# Autodesk Inventor assembly: NASA-20-EBOX-EXT-01
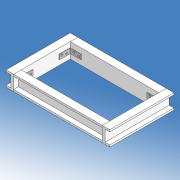
[picture p0: Inventor's stored thumbnail of the model, 180x180]
Saved by Autodesk Inventor 2020 (Build 240168000, 168)
## iProperties
Created: 2019-10-09
Part Number: NASA-20-EBOX-EXT-01
Document SubType Name: Assembly
Designer: mpark
Author: mpark
## Documents named in this file (4)
- C:\Users\mpark\Documents\NASA20\Inventor Files\NASA-20\NASA-20\E-Box\NASA-20-EBOX-EXT-01.iam
- C:\Users\mpark\Documents\NASA20\Inventor Files\NASA-20\NASA-20\E-Box\NASA-20-EBOX-EXTC-01.ipt
- C:\Users\mpark\Documents\NASA20\Inventor Files\NASA-20\NASA-20\E-Box\NASA-20-EBOX-SEXTC-01.ipt
- C:\Users\mpark\Documents\NASA20\Inventor Files\NASA-20\NASA-20\E-Box\1556A630_BRACKET.ipt
## Components (8 placed, 3 different names)
1. NASA-20-EBOX-EXTC-01:1 — Flush:1, Flush:2, Flush:5, Mate:1, Mate:2, Flush:8, Mate:8, Mate:9, Flush:9
2. NASA-20-EBOX-EXTC-01:2 — Flush:1, Flush:2, Flush:3, Flush:4, Flush:5, Flush:6, Flush:7, Mate:11, Mate:12
3. NASA-20-EBOX-SEXTC-01:1 — Flush:4, Mate:2, Flush:7, Mate:3, Mate:13
4. NASA-20-EBOX-SEXTC-01:2 — Flush:3, Mate:1, Flush:6, Flush:8, Mate:4, Mate:10
5. 1556A630_BRACKET:1 — Mate:3, Mate:8, Flush:9, Flush:10, Flush:11
6. 1556A630_BRACKET:4 — Mate:4, Mate:9, Flush:10
7. 1556A630_BRACKET:5 — Mate:10, Mate:11, Flush:12
8. 1556A630_BRACKET:6 — Mate:12, Mate:13, Flush:11, Flush:12
## Relationships (22: Flush 12, Mate 10)
- Flush:1: NASA-20-EBOX-EXTC-01:1 ↔ NASA-20-EBOX-EXTC-01:2
- Flush:2: NASA-20-EBOX-EXTC-01:1 ↔ NASA-20-EBOX-EXTC-01:2
- Flush:3: NASA-20-EBOX-EXTC-01:2 ↔ NASA-20-EBOX-SEXTC-01:2
- Flush:4: NASA-20-EBOX-EXTC-01:2 ↔ NASA-20-EBOX-SEXTC-01:1
- Flush:5: NASA-20-EBOX-EXTC-01:1 ↔ NASA-20-EBOX-EXTC-01:2
- Mate:1: NASA-20-EBOX-EXTC-01:1 ↔ NASA-20-EBOX-SEXTC-01:2
- Mate:2: NASA-20-EBOX-EXTC-01:1 ↔ NASA-20-EBOX-SEXTC-01:1
- Flush:6: NASA-20-EBOX-EXTC-01:2 ↔ NASA-20-EBOX-SEXTC-01:2
- Flush:7: NASA-20-EBOX-EXTC-01:2 ↔ NASA-20-EBOX-SEXTC-01:1
- Flush:8: NASA-20-EBOX-EXTC-01:1 ↔ NASA-20-EBOX-SEXTC-01:2
- Mate:3: NASA-20-EBOX-SEXTC-01:1 ↔ 1556A630_BRACKET:1
- Mate:4: NASA-20-EBOX-SEXTC-01:2 ↔ 1556A630_BRACKET:4
- Mate:8: NASA-20-EBOX-EXTC-01:1 ↔ 1556A630_BRACKET:1
- Mate:9: NASA-20-EBOX-EXTC-01:1 ↔ 1556A630_BRACKET:4
- Mate:10: NASA-20-EBOX-SEXTC-01:2 ↔ 1556A630_BRACKET:5
- Mate:11: NASA-20-EBOX-EXTC-01:2 ↔ 1556A630_BRACKET:5
- Flush:9 (17.4625 mm): NASA-20-EBOX-EXTC-01:1 ↔ 1556A630_BRACKET:1
- Flush:10: 1556A630_BRACKET:1 ↔ 1556A630_BRACKET:4
- Mate:12: NASA-20-EBOX-EXTC-01:2 ↔ 1556A630_BRACKET:6
- Mate:13: NASA-20-EBOX-SEXTC-01:1 ↔ 1556A630_BRACKET:6
- Flush:11: 1556A630_BRACKET:1 ↔ 1556A630_BRACKET:6
- Flush:12: 1556A630_BRACKET:5 ↔ 1556A630_BRACKET:6
